# Autodesk Inventor assembly: Transformador
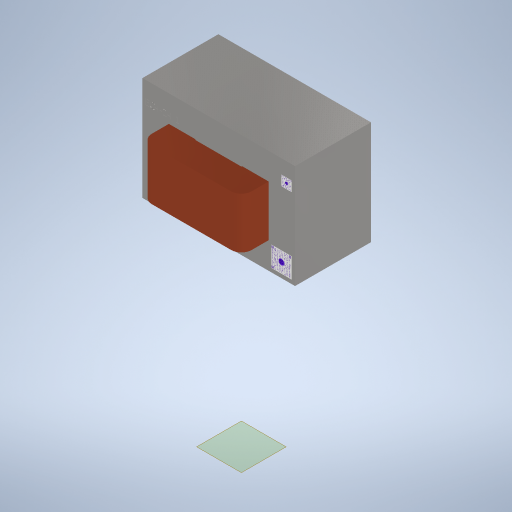
[picture p0: Inventor's stored thumbnail of the model, 512x512]
Saved by Autodesk Inventor 2024.2 (Build 282272000, 272)
## iProperties
Created: 2024-05-06
Part Number: Transformador
Document SubType Name: Assembly
Designer: 082220019
Author: 082220019
## Documents named in this file (4)
- C:\Users\082220019\Downloads\PBL-EC4-24-1-main (1)\PBL-EC4-24-1-main\Transformador.iam
- C:\Users\082220019\Downloads\PBL-EC4-24-1-main (1)\PBL-EC4-24-1-main\Fechamento.ipt
- C:\Users\082220019\Downloads\PBL-EC4-24-1-main (1)\PBL-EC4-24-1-main\Chapa.ipt
- C:\Users\082220019\Downloads\PBL-EC4-24-1-main (1)\PBL-EC4-24-1-main\Bobina.ipt
## Components (211 placed, 3 different names)
1. Bobina:1
2. Chapa:1 — Mate:1, Flush:1, Flush:2
3. Fechamento:1 — Mate:1, Flush:1, Flush:2
4. Chapa:2
5. Fechamento:2
6. Chapa:3
7. Fechamento:3
8. Chapa:4
9. Fechamento:4
10. Chapa:5
11. Fechamento:5
12. Chapa:6
13. Fechamento:6
14. Chapa:7
15. Fechamento:7
16. Chapa:8
17. Fechamento:8
18. Chapa:9
19. Fechamento:9
20. Chapa:10
21. Fechamento:10
22. Chapa:11
23. Fechamento:11
24. Chapa:12
25. Fechamento:12
26. Chapa:13
27. Fechamento:13
28. Chapa:14
29. Fechamento:14
30. Chapa:15
31. Fechamento:15
32. Chapa:16
33. Fechamento:16
34. Chapa:17
35. Fechamento:17
36. Chapa:18
37. Fechamento:18
38. Chapa:19
39. Fechamento:19
40. Chapa:20
41. Fechamento:20
42. Chapa:21
43. Fechamento:21
44. Chapa:22
45. Fechamento:22
46. Chapa:23
47. Fechamento:23
48. Chapa:24
49. Fechamento:24
50. Chapa:25
51. Fechamento:25
52. Chapa:26
53. Fechamento:26
54. Chapa:27
55. Fechamento:27
56. Chapa:28
57. Fechamento:28
58. Chapa:29
59. Fechamento:29
60. Chapa:30
61. Fechamento:30
62. Chapa:31
63. Fechamento:31
64. Chapa:32
65. Fechamento:32
66. Chapa:33
67. Fechamento:33
68. Chapa:34
69. Fechamento:34
70. Chapa:35
71. Fechamento:35
72. Chapa:36
73. Fechamento:36
74. Chapa:37
75. Fechamento:37
76. Chapa:38
77. Fechamento:38
78. Chapa:39
79. Fechamento:39
80. Chapa:40
81. Fechamento:40
82. Chapa:41
83. Fechamento:41
84. Chapa:42
85. Fechamento:42
86. Chapa:43
87. Fechamento:43
88. Chapa:44
89. Fechamento:44
90. Chapa:45
91. Fechamento:45
92. Chapa:46
93. Fechamento:46
94. Chapa:47
95. Fechamento:47
96. Chapa:48
97. Fechamento:48
98. Chapa:49
99. Fechamento:49
100. Chapa:50
101. Fechamento:50
102. Chapa:51
103. Fechamento:51
104. Chapa:52
105. Fechamento:52
106. Chapa:53
107. Fechamento:53
108. Chapa:54
109. Fechamento:54
110. Chapa:55
111. Fechamento:55
112. Chapa:56
113. Fechamento:56
114. Chapa:57
115. Fechamento:57
116. Chapa:58
117. Fechamento:58
118. Chapa:59
119. Fechamento:59
120. Chapa:60
121. Fechamento:60
122. Chapa:61
123. Fechamento:61
124. Chapa:62
125. Fechamento:62
126. Chapa:63
127. Fechamento:63
128. Chapa:64
129. Fechamento:64
130. Chapa:65
131. Fechamento:65
132. Chapa:66
133. Fechamento:66
134. Chapa:67
135. Fechamento:67
136. Chapa:68
137. Fechamento:68
138. Chapa:69
139. Fechamento:69
140. Chapa:70
141. Fechamento:70
142. Chapa:71
143. Fechamento:71
144. Chapa:72
145. Fechamento:72
146. Chapa:73
147. Fechamento:73
148. Chapa:74
149. Fechamento:74
150. Chapa:75
151. Fechamento:75
152. Chapa:76
153. Fechamento:76
154. Chapa:77
155. Fechamento:77
156. Chapa:78
157. Fechamento:78
158. Chapa:79
159. Fechamento:79
160. Chapa:80
161. Fechamento:80
162. Chapa:81
163. Fechamento:81
164. Chapa:82
165. Fechamento:82
166. Chapa:83
167. Fechamento:83
168. Chapa:84
169. Fechamento:84
170. Chapa:85
171. Fechamento:85
172. Chapa:86
173. Fechamento:86
174. Chapa:87
175. Fechamento:87
176. Chapa:88
177. Fechamento:88
178. Chapa:89
179. Fechamento:89
180. Chapa:90
181. Fechamento:90
182. Chapa:91
183. Fechamento:91
184. Chapa:92
185. Fechamento:92
186. Chapa:93
187. Fechamento:93
188. Chapa:94
189. Fechamento:94
190. Chapa:95
191. Fechamento:95
192. Chapa:96
193. Fechamento:96
194. Chapa:97
195. Fechamento:97
196. Chapa:98
197. Fechamento:98
198. Chapa:99
199. Fechamento:99
200. Chapa:100
201. Fechamento:100
202. Chapa:101
203. Fechamento:101
204. Chapa:102
205. Fechamento:102
206. Chapa:103
207. Fechamento:103
208. Chapa:104
209. Fechamento:104
210. Chapa:105
211. Fechamento:105
## Component patterns: (105 elements, first: Chapa:1 + Fechamento:1)
## Relationships (3: Flush 2, Mate 1)
- Mate:1: Chapa:1 ↔ Fechamento:1
- Flush:1: Chapa:1 ↔ Fechamento:1
- Flush:2: Chapa:1 ↔ Fechamento:1
